# Autodesk Inventor assembly: PNAP-Assembly
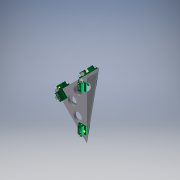
[picture p0: Inventor's stored thumbnail of the model, 180x180]
Saved by Autodesk Inventor 2016 (Build 200138000, 138)
## iProperties
Created: 2016-07-01
Part Number: PNAP-Assembly
Document SubType Name: Assembly
Designer: kam42
Author: kam42
## Documents named in this file (4)
- C:\Users\kam42\Documents\Git Repos\duke-pnap\PNAP-Assembly.iam
- C:\Users\kam42\Documents\Git Repos\duke-pnap\PNAP Mount temp\Part2-01.ipt
- C:\Users\kam42\Documents\Git Repos\duke-pnap\PNAP Mount temp.ipt
- C:\Users\kam42\Documents\Git Repos\duke-pnap\Sensor Models\Endevco-7264D\Endevco-7264D.ipt
## Components (10 placed, 2 different names)
1. Part2-01:1 — Mate:1, Mate:2, Mate:3, Mate:4, Mate:5, Mate:6, Mate:7, Mate:8, Mate:9, Mate:10, Angle:1
2. Endevco-7264D:1 — Mate:1, Mate:4, Mate:7
3. Endevco-7264D:2 — Mate:2, Mate:8, Mate:9
4. Endevco-7264D:3 — Mate:3, Mate:5, Mate:6
5. Endevco-7264D:4
6. Endevco-7264D:5
7. Endevco-7264D:6
8. Endevco-7264D:7
9. Endevco-7264D:8
10. Endevco-7264D:9
## Component patterns: (3 elements, first: Endevco-7264D:1 + Endevco-7264D:2 + Endevco-7264D:3)
## Relationships (11: Mate 10, Angle 1)
- Mate:1: Part2-01:1 ↔ Endevco-7264D:1
- Mate:2: Part2-01:1 ↔ Endevco-7264D:2
- Mate:3: Part2-01:1 ↔ Endevco-7264D:3
- Mate:4: Part2-01:1 ↔ Endevco-7264D:1
- Mate:5: Part2-01:1 ↔ Endevco-7264D:3
- Mate:6: Part2-01:1 ↔ Endevco-7264D:3
- Mate:7: Part2-01:1 ↔ Endevco-7264D:1
- Mate:8: Part2-01:1 ↔ Endevco-7264D:2
- Mate:9: Part2-01:1 ↔ Endevco-7264D:2
- Mate:10: Part2-01:1
- Angle:1 (0 deg): Part2-01:1
